# Autodesk Inventor assembly: covered motor
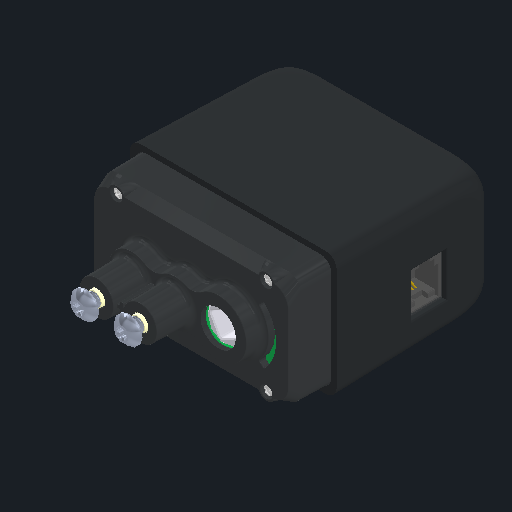
[picture p0: Inventor's stored thumbnail of the model, 512x512]
Saved by Autodesk Inventor 2024 (Build 280153000, 153)
## iProperties
Created: 2024-01-04
Part Number: covered motor
Document SubType Name: Assembly
Designer: macbook
Author: macbook
## Documents named in this file (3)
- \\Mac\Home\Desktop\code\1599V-VRC\Cad\Assembly\covered motor - Copy.iam
- \\Mac\Home\Desktop\code\1599V-VRC\Cad\Assembly\thick screw motor.iam
- \\Mac\Home\Desktop\code\1599V-VRC\Cad\Assembly\motor cover.ipt
## Components (2 placed, 2 different names)
1. thick screw motor:1 [sub-assembly]
2. motor cover:1
## Relationships (3: Mate 3)
- [Mate]: thick screw motor:1 ↔ motor cover:1
- [Mate]: thick screw motor:1 ↔ motor cover:1
- [Mate]: thick screw motor:1 ↔ motor cover:1
